# Autodesk Inventor assembly: Traveler Assya
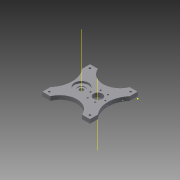
[picture p0: Inventor's stored thumbnail of the model, 180x180]
Saved by Autodesk Inventor 2015 (Build 190159000, 159)
## iProperties
Created: 2015-01-23
Part Number: Traveler Assya
Document SubType Name: Assembly
Designer: chappelled
Author: chappelled
## Documents named in this file (7)
- \\lhssvr02\Homedirs\Robotics Club\Hardware & CAD\CAD Model 2015\Claw Doug\Traveler Assya.iam
- \\lhssvr02\Homedirs\Robotics Club\Hardware & CAD\CAD Model 2015\Claw Doug\Traveler.ipt
- C:\Users\chappelled\Documents\Inventor\Content Center Files\R2014\en-US\ASME B18.21.1(02)\ASME B18.21.1 - 1_4 Extra-Duty. Lock Washers (Inch Series)Extra-Duty Helical Spring Lock Washer(7).ipt
- C:\Users\chappelled\Documents\Inventor\Content Center Files\R2014\en-US\IFI 100 107(2)\IFI 100_107 - 1_4 - 20 Metal Type.ipt
- C:\Users\chappelled\Documents\Inventor\Content Center Files\R2014\en-US\ANSI B27.7M\ANSI B27.7M - 3CMI-15.ipt
- \\lhssvr02\Homedirs\Robotics Club\Hardware & CAD\CAD Model 2015\Claw Doug\Traveler Assy\Design Accelerator\Bolted Connection4.iam
- \\lhssvr02\Homedirs\Robotics Club\Hardware & CAD\CAD Model 2015\Claw Doug\Traveler Assy\Design Accelerator\Bolted Connection6.iam
## Components (6 placed, 5 different names)
1. Traveler:1 — Mate:31, Mate:44, Mate:45, Mate:46, Mate:47
2. Extra-Duty Helical Spring Lock Washer (Inch) 1/4 Extra-Duty. Lock Washers (Inch Series)Extra-Duty Helical Spring Lock Washer:1 — Mate:39
3. Prevailing Torque Type Hex Nut - Inch (IFI) 1/4 - 20 Metal Type:1 — Mate:39
4. ANSI B27.7M 3CMI-15:1
5. Bolted Connection:1 [sub-assembly] — Mate:46, Mate:47
6. Bolted Connection:2 [sub-assembly] — Mate:44, Mate:45
## Relationships (8: Mate 8)
- Mate:30
- Mate:31: Traveler:1
- Mate:35
- Mate:39: Extra-Duty Helical Spring Lock Washer (Inch) 1/4 Extra-Duty. Lock Washers (Inch Series)Extra-Duty Helical Spring Lock Washer:1 ↔ Prevailing Torque Type Hex Nut - Inch (IFI) 1/4 - 20 Metal Type:1
- Mate:44: Traveler:1 ↔ Bolted Connection:2
- Mate:45: Traveler:1 ↔ Bolted Connection:2
- Mate:46: Traveler:1 ↔ Bolted Connection:1
- Mate:47: Traveler:1 ↔ Bolted Connection:1
